# Autodesk Inventor assembly: ASY MSC 800 gills
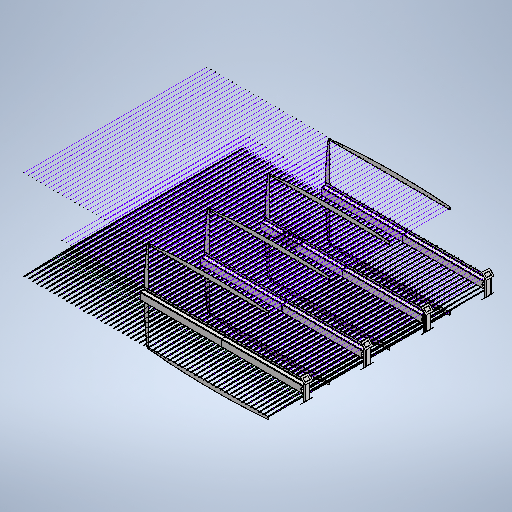
[picture p0: Inventor's stored thumbnail of the model, 512x512]
Saved by Autodesk Inventor 2025.1 (Build 291241020, 241B)
## iProperties
Created: 2024-08-31
Part Number: ASY MSC 800 gills
Document SubType Name: Assembly
Designer: pokla
Stock Number: ASY МОО 800 Жабры
Mass: 469810 g
Surface Area: 1.86943e+06 cm^2
Volume: 67870.7 cm^3
Density: 6.92212 g/cm^3
Author: pokla
## Documents named in this file (14)
- C:\Users\user\YandexDisk-badmisterfox\домашниий пк\Inventor\Manturovo\Manturovo_Se-clar\ASY MSC 800 gills.iam
- C:\Users\user\YandexDisk-badmisterfox\домашниий пк\Inventor\Manturovo\Manturovo_Se-clar\MSC 804 sheet gills.ipt
- C:\Users\user\YandexDisk-badmisterfox\домашниий пк\Inventor\Manturovo\Manturovo_Se-clar\MSC 810 pillar gills.ipt
- C:\Users\user\YandexDisk-badmisterfox\домашниий пк\Inventor\Manturovo\Manturovo_Se-clar\MSC 805 sheet gills.ipt
- C:\Users\user\YandexDisk-badmisterfox\домашниий пк\Inventor\Manturovo\Manturovo_Se-clar\MSC 806 sheet gills.ipt
- C:\Users\user\YandexDisk-badmisterfox\домашниий пк\Inventor\Manturovo\Manturovo_Se-clar\MSC 807 sheet gills.ipt
- C:\Users\user\YandexDisk-badmisterfox\домашниий пк\Inventor\Manturovo\Manturovo_Se-clar\MSC 808 sheet gills.ipt
- C:\Users\user\YandexDisk-badmisterfox\домашниий пк\Inventor\Manturovo\Manturovo_Se-clar\MSC 809 sheet gills.ipt
- C:\Users\user\YandexDisk-badmisterfox\домашниий пк\Inventor\Manturovo\Manturovo_Se-clar\MSC 813 wall support gills.ipt
- C:\Users\user\YandexDisk-badmisterfox\домашниий пк\Inventor\Manturovo\Manturovo_Se-clar\MSC 811 pillar gills.ipt
- C:\Users\user\YandexDisk-badmisterfox\домашниий пк\Inventor\Manturovo\Manturovo_Se-clar\MSC 814 string for sheets gills.ipt
- C:\Users\user\YandexDisk-badmisterfox\домашниий пк\Inventor\Manturovo\Manturovo_Se-clar\MSC 812 top support gills.ipt
- C:\Users\user\YandexDisk-badmisterfox\домашниий пк\Inventor\Manturovo\Manturovo_Se-clar\MSC 803 sheet gills.ipt
- C:\Users\user\YandexDisk-badmisterfox\домашниий пк\Inventor\Manturovo\Manturovo_Se-clar\ASY MSC 800.1 gills base.iam
## Components (393 placed, 13 different names)
1. MSC 0203 sheet gills:1 — Angle:2, Tangent:8, Tangent:9, Flush:15, Flush:19
2. MSC 0204 sheet gills:1 — Angle:3, Tangent:10, Tangent:11, Flush:15, Flush:16
3. MSC 0205 sheet gills:1 — Angle:4, Tangent:12, Tangent:13, Flush:16, Flush:17
4. MSC 0206 sheet gills:1 — Angle:5, Tangent:17, Tangent:18, Flush:17, Flush:18
5. MSC 0207 sheet gills:1 — Angle:6, Tangent:19, Tangent:20, Flush:18
6. MSC 814 string for sheets gills:143 — Rigid:40
7. MSC 0203 sheet gills:2
8. MSC 0204 sheet gills:2
9. MSC 0205 sheet gills:2
10. MSC 0206 sheet gills:2
11. MSC 0207 sheet gills:2
12. MSC 814 string for sheets gills:152 — Rigid:24
13. MSC 814 string for sheets gills:371
14. MSC 814 string for sheets gills:372
15. MSC 814 string for sheets gills:373
16. MSC 814 string for sheets gills:374
17. MSC 814 string for sheets gills:375
18. MSC 814 string for sheets gills:2 — Rigid:12
19. MSC 0201 sheet gills:1 — Rigid:33, Angle:2, Angle:3, Angle:4, Angle:5, Angle:6, Tangent:14, Tangent:15, Tangent:16, Flush:19
20. MSC 804 sheet gills:1 — Rigid:33
21. MSC 814 string for sheets gills:1 — Rotational:1
22. MSC 814 string for sheets gills:3 — Rotational:2
23. MSC 814 string for sheets gills:376 — Rotational:3
24. MSC 814 string for sheets gills:377
25. MSC 0201 sheet gills:2
26. MSC 804 sheet gills:2
27. MSC 814 string for sheets gills:378
28. MSC 814 string for sheets gills:379
29. MSC 814 string for sheets gills:380
30. MSC 814 string for sheets gills:381
31. MSC 0201 sheet gills:3
32. MSC 804 sheet gills:3
33. MSC 814 string for sheets gills:382
34. MSC 814 string for sheets gills:383
35. MSC 814 string for sheets gills:384
36. MSC 814 string for sheets gills:385
37. MSC 0201 sheet gills:4
38. MSC 804 sheet gills:4
39. MSC 814 string for sheets gills:386
40. MSC 814 string for sheets gills:387
41. MSC 814 string for sheets gills:388
42. MSC 814 string for sheets gills:389
43. MSC 0201 sheet gills:5
44. MSC 804 sheet gills:5
45. MSC 814 string for sheets gills:390
46. MSC 814 string for sheets gills:391
47. MSC 814 string for sheets gills:392
48. MSC 814 string for sheets gills:393
49. MSC 0201 sheet gills:6
50. MSC 804 sheet gills:6
51. MSC 814 string for sheets gills:394
52. MSC 814 string for sheets gills:395
53. MSC 814 string for sheets gills:396
54. MSC 814 string for sheets gills:397
55. MSC 0201 sheet gills:7
56. MSC 804 sheet gills:7
57. MSC 814 string for sheets gills:398
58. MSC 814 string for sheets gills:399
59. MSC 814 string for sheets gills:400
60. MSC 814 string for sheets gills:401
61. MSC 0201 sheet gills:8
62. MSC 804 sheet gills:8
63. MSC 814 string for sheets gills:402
64. MSC 814 string for sheets gills:403
65. MSC 814 string for sheets gills:404
66. MSC 814 string for sheets gills:405
67. MSC 0201 sheet gills:9
68. MSC 804 sheet gills:9
69. MSC 814 string for sheets gills:406
70. MSC 814 string for sheets gills:407
71. MSC 814 string for sheets gills:408
72. MSC 814 string for sheets gills:409
73. MSC 0201 sheet gills:10
74. MSC 804 sheet gills:10
75. MSC 814 string for sheets gills:410
76. MSC 814 string for sheets gills:411
77. MSC 814 string for sheets gills:412
78. MSC 814 string for sheets gills:413
79. MSC 0201 sheet gills:11
80. MSC 804 sheet gills:11
81. MSC 814 string for sheets gills:414
82. MSC 814 string for sheets gills:415
83. MSC 814 string for sheets gills:416
84. MSC 814 string for sheets gills:417
85. MSC 0201 sheet gills:12
86. MSC 804 sheet gills:12
87. MSC 814 string for sheets gills:418
88. MSC 814 string for sheets gills:419
89. MSC 814 string for sheets gills:420
90. MSC 814 string for sheets gills:421
91. MSC 0201 sheet gills:13
92. MSC 804 sheet gills:13
93. MSC 814 string for sheets gills:422
94. MSC 814 string for sheets gills:423
95. MSC 814 string for sheets gills:424
96. MSC 814 string for sheets gills:425
97. MSC 0201 sheet gills:14
98. MSC 804 sheet gills:14
99. MSC 814 string for sheets gills:426
100. MSC 814 string for sheets gills:427
101. MSC 814 string for sheets gills:428
102. MSC 814 string for sheets gills:429
103. MSC 0201 sheet gills:15
104. MSC 804 sheet gills:15
105. MSC 814 string for sheets gills:430
106. MSC 814 string for sheets gills:431
107. MSC 814 string for sheets gills:432
108. MSC 814 string for sheets gills:433
109. MSC 0201 sheet gills:16
110. MSC 804 sheet gills:16
111. MSC 814 string for sheets gills:434
112. MSC 814 string for sheets gills:435
113. MSC 814 string for sheets gills:436
114. MSC 814 string for sheets gills:437
115. MSC 0201 sheet gills:17
116. MSC 804 sheet gills:17
117. MSC 814 string for sheets gills:438
118. MSC 814 string for sheets gills:439
119. MSC 814 string for sheets gills:440
120. MSC 814 string for sheets gills:441
121. MSC 0201 sheet gills:18
122. MSC 804 sheet gills:18
123. MSC 814 string for sheets gills:442
124. MSC 814 string for sheets gills:443
125. MSC 814 string for sheets gills:444
126. MSC 814 string for sheets gills:445
127. MSC 0201 sheet gills:19
128. MSC 804 sheet gills:19
129. MSC 814 string for sheets gills:446
130. MSC 814 string for sheets gills:447
131. MSC 814 string for sheets gills:448
132. MSC 814 string for sheets gills:449
133. MSC 0201 sheet gills:20
134. MSC 804 sheet gills:20
135. MSC 814 string for sheets gills:450
136. MSC 814 string for sheets gills:451
137. MSC 814 string for sheets gills:452
138. MSC 814 string for sheets gills:453
139. MSC 0201 sheet gills:21
140. MSC 804 sheet gills:21
141. MSC 814 string for sheets gills:454
142. MSC 814 string for sheets gills:455
143. MSC 814 string for sheets gills:456
144. MSC 814 string for sheets gills:457
145. MSC 0201 sheet gills:22
146. MSC 804 sheet gills:22
147. MSC 814 string for sheets gills:458
148. MSC 814 string for sheets gills:459
149. MSC 814 string for sheets gills:460
150. MSC 814 string for sheets gills:461
151. MSC 0201 sheet gills:23
152. MSC 804 sheet gills:23
153. MSC 814 string for sheets gills:462
154. MSC 814 string for sheets gills:463
155. MSC 814 string for sheets gills:464
156. MSC 814 string for sheets gills:465
157. MSC 0201 sheet gills:24
158. MSC 804 sheet gills:24
159. MSC 814 string for sheets gills:466
160. MSC 814 string for sheets gills:467
161. MSC 814 string for sheets gills:468
162. MSC 814 string for sheets gills:469
163. MSC 0201 sheet gills:25
164. MSC 804 sheet gills:25
165. MSC 814 string for sheets gills:470
166. MSC 814 string for sheets gills:471
167. MSC 814 string for sheets gills:472
168. MSC 814 string for sheets gills:473
169. MSC 0201 sheet gills:26
170. MSC 804 sheet gills:26
171. MSC 814 string for sheets gills:474
172. MSC 814 string for sheets gills:475
173. MSC 814 string for sheets gills:476
174. MSC 814 string for sheets gills:477
175. MSC 0201 sheet gills:27
176. MSC 804 sheet gills:27
177. MSC 814 string for sheets gills:478
178. MSC 814 string for sheets gills:479
179. MSC 814 string for sheets gills:480
180. MSC 814 string for sheets gills:481
181. MSC 0201 sheet gills:28
182. MSC 804 sheet gills:28
183. MSC 814 string for sheets gills:482
184. MSC 814 string for sheets gills:483
185. MSC 814 string for sheets gills:484
186. MSC 814 string for sheets gills:485
187. MSC 0201 sheet gills:29
188. MSC 804 sheet gills:29
189. MSC 814 string for sheets gills:486
190. MSC 814 string for sheets gills:487
191. MSC 814 string for sheets gills:488
192. MSC 814 string for sheets gills:489
193. MSC 0201 sheet gills:30
194. MSC 804 sheet gills:30
195. MSC 814 string for sheets gills:490
196. MSC 814 string for sheets gills:491
197. MSC 814 string for sheets gills:492
198. MSC 814 string for sheets gills:493
199. MSC 0201 sheet gills:31
200. MSC 804 sheet gills:31
201. MSC 814 string for sheets gills:494
202. MSC 814 string for sheets gills:495
203. MSC 814 string for sheets gills:496
204. MSC 814 string for sheets gills:497
205. MSC 0201 sheet gills:32
206. MSC 804 sheet gills:32
207. MSC 814 string for sheets gills:498
208. MSC 814 string for sheets gills:499
209. MSC 814 string for sheets gills:500
210. MSC 814 string for sheets gills:501
211. MSC 0201 sheet gills:33
212. MSC 804 sheet gills:33
213. MSC 814 string for sheets gills:502
214. MSC 814 string for sheets gills:503
215. MSC 814 string for sheets gills:504
216. MSC 814 string for sheets gills:505
217. MSC 0201 sheet gills:34
218. MSC 804 sheet gills:34
219. MSC 814 string for sheets gills:506
220. MSC 814 string for sheets gills:507
221. MSC 814 string for sheets gills:508
222. MSC 814 string for sheets gills:509
223. MSC 0201 sheet gills:35
224. MSC 804 sheet gills:35
225. MSC 814 string for sheets gills:510
226. MSC 814 string for sheets gills:511
227. MSC 814 string for sheets gills:512
228. MSC 814 string for sheets gills:513
229. MSC 0201 sheet gills:36
230. MSC 804 sheet gills:36
231. MSC 814 string for sheets gills:514
232. MSC 814 string for sheets gills:515
233. MSC 814 string for sheets gills:516
234. MSC 814 string for sheets gills:517
235. MSC 0201 sheet gills:37
236. MSC 804 sheet gills:37
237. MSC 814 string for sheets gills:518
238. MSC 814 string for sheets gills:519
239. MSC 814 string for sheets gills:520
240. MSC 814 string for sheets gills:521
241. MSC 0201 sheet gills:38
242. MSC 804 sheet gills:38
243. MSC 814 string for sheets gills:522
244. MSC 814 string for sheets gills:523
245. MSC 814 string for sheets gills:524
246. MSC 814 string for sheets gills:525
247. MSC 0201 sheet gills:39
248. MSC 804 sheet gills:39
249. MSC 814 string for sheets gills:526
250. MSC 814 string for sheets gills:527
251. MSC 814 string for sheets gills:528
252. MSC 814 string for sheets gills:529
253. MSC 0201 sheet gills:40
254. MSC 804 sheet gills:40
255. MSC 814 string for sheets gills:530
256. MSC 814 string for sheets gills:531
257. MSC 814 string for sheets gills:532
258. MSC 814 string for sheets gills:533
259. MSC 0201 sheet gills:41
260. MSC 804 sheet gills:41
261. MSC 814 string for sheets gills:534
262. MSC 814 string for sheets gills:535
263. MSC 814 string for sheets gills:536
264. MSC 814 string for sheets gills:537
265. MSC 0201 sheet gills:42
266. MSC 804 sheet gills:42
267. MSC 814 string for sheets gills:538
268. MSC 814 string for sheets gills:539
269. MSC 814 string for sheets gills:540
270. MSC 814 string for sheets gills:541
271. MSC 0201 sheet gills:43
272. MSC 804 sheet gills:43
273. MSC 814 string for sheets gills:542
274. MSC 814 string for sheets gills:543
275. MSC 814 string for sheets gills:544
276. MSC 814 string for sheets gills:545
277. MSC 0201 sheet gills:44
278. MSC 804 sheet gills:44
279. MSC 814 string for sheets gills:546
280. MSC 814 string for sheets gills:547
281. MSC 814 string for sheets gills:548
282. MSC 814 string for sheets gills:549
283. MSC 0201 sheet gills:45
284. MSC 804 sheet gills:45
285. MSC 814 string for sheets gills:550
286. MSC 814 string for sheets gills:551
287. MSC 814 string for sheets gills:552
288. MSC 814 string for sheets gills:553
289. MSC 0201 sheet gills:46
290. MSC 804 sheet gills:46
291. MSC 814 string for sheets gills:554
292. MSC 814 string for sheets gills:555
293. MSC 814 string for sheets gills:556
294. MSC 814 string for sheets gills:557
295. MSC 0201 sheet gills:47
296. MSC 804 sheet gills:47
297. MSC 814 string for sheets gills:558
298. MSC 814 string for sheets gills:559
299. MSC 814 string for sheets gills:560
300. MSC 814 string for sheets gills:561
301. MSC 0201 sheet gills:48
302. MSC 804 sheet gills:48
303. MSC 814 string for sheets gills:562
304. MSC 814 string for sheets gills:563
305. MSC 814 string for sheets gills:564
306. MSC 814 string for sheets gills:565
307. MSC 0201 sheet gills:49
308. MSC 804 sheet gills:49
309. MSC 814 string for sheets gills:566
310. MSC 814 string for sheets gills:567
311. MSC 814 string for sheets gills:568
312. MSC 814 string for sheets gills:569
313. MSC 0201 sheet gills:50
314. MSC 804 sheet gills:50
315. MSC 814 string for sheets gills:570
316. MSC 814 string for sheets gills:571
317. MSC 814 string for sheets gills:572
318. MSC 814 string for sheets gills:573
319. MSC 0201 sheet gills:51
320. MSC 804 sheet gills:51
321. MSC 814 string for sheets gills:574
322. MSC 814 string for sheets gills:575
323. MSC 814 string for sheets gills:576
324. MSC 814 string for sheets gills:577
325. MSC 0201 sheet gills:52
326. MSC 804 sheet gills:52
327. MSC 814 string for sheets gills:578
328. MSC 814 string for sheets gills:579
329. MSC 814 string for sheets gills:580
330. MSC 814 string for sheets gills:581
331. MSC 0201 sheet gills:53
332. MSC 804 sheet gills:53
333. MSC 814 string for sheets gills:582
334. MSC 814 string for sheets gills:583
335. MSC 814 string for sheets gills:584
336. MSC 814 string for sheets gills:585
337. MSC 0201 sheet gills:54
338. MSC 804 sheet gills:54
339. MSC 814 string for sheets gills:586
340. MSC 814 string for sheets gills:587
341. MSC 814 string for sheets gills:588
342. MSC 814 string for sheets gills:589
343. MSC 0201 sheet gills:55
344. MSC 804 sheet gills:55
345. MSC 814 string for sheets gills:590
346. MSC 814 string for sheets gills:591
347. MSC 814 string for sheets gills:592
348. MSC 814 string for sheets gills:593
349. MSC 0201 sheet gills:56
350. MSC 804 sheet gills:56
351. MSC 814 string for sheets gills:594
352. MSC 814 string for sheets gills:595
353. MSC 814 string for sheets gills:596
354. MSC 814 string for sheets gills:597
355. MSC 0201 sheet gills:57
356. MSC 804 sheet gills:57
357. MSC 814 string for sheets gills:598
358. MSC 814 string for sheets gills:599
359. MSC 814 string for sheets gills:600
360. MSC 814 string for sheets gills:601
361. MSC 0201 sheet gills:58
362. MSC 804 sheet gills:58
363. MSC 814 string for sheets gills:602
364. MSC 814 string for sheets gills:603
365. MSC 814 string for sheets gills:604
366. MSC 813 wall support gills:1 — Rigid:12, Rigid:30, Tangent:14, Tangent:15
367. MSC 812 top support gills:1 — Rigid:28, Rigid:30, Tangent:8, Tangent:9, Tangent:10, Tangent:11, Tangent:12, Tangent:13, Tangent:17, Tangent:18, Tangent:19, Tangent:20, Rigid:40
368. MSC 811 pillar gills:1 — Rigid:28, Rigid:29
369. MSC 812 top support gills:2 — Rigid:24, Rigid:29, Rigid:31
370. MSC 813 wall support gills:2 — Rigid:31, Rotational:3
371. MSC 810 pillar gills:1 — Rotational:1, Rotational:2, Tangent:16
372. ASY MSC 800.1 gills base:1 [sub-assembly]
373. MSC 813 wall support gills:4
374. MSC 812 top support gills:3
375. MSC 811 pillar gills:2
376. MSC 812 top support gills:4
377. MSC 813 wall support gills:5
378. MSC 810 pillar gills:2
379. ASY MSC 800.1 gills base:2 [sub-assembly]
380. MSC 813 wall support gills:6
381. MSC 812 top support gills:5
382. MSC 811 pillar gills:3
383. MSC 812 top support gills:6
384. MSC 813 wall support gills:7
385. MSC 810 pillar gills:3
386. ASY MSC 800.1 gills base:3 [sub-assembly]
387. MSC 813 wall support gills:8
388. MSC 812 top support gills:7
389. MSC 811 pillar gills:4
390. MSC 812 top support gills:8
391. MSC 813 wall support gills:9
392. MSC 810 pillar gills:4
393. ASY MSC 800.1 gills base:4 [sub-assembly]
## Component patterns: (6 elements, first: MSC 814 string for sheets gills:152), (58 elements, first: MSC 814 string for sheets gills:2 + MSC 0201 sheet gills:1 + MSC 804 sheet gills:1 + MSC 814 string for sheets gills:1 + MSC 814 string for sheets gills:3 + MSC 814 string for sheets gills:376), (4 elements, first: MSC 813 wall support gills:1 + MSC 812 top support gills:1 + MSC 811 pillar gills:1 + MSC 812 top support gills:2 + MSC 813 wall support gills:2 + MSC 810 pillar gills:1 + ASY MSC 800.1 gills base:1)
## Relationships (45: Tangent 13, Flush 12, WeldJoint 9, Angle 5, Mate 3, RevoluteJoint 3)
- [WeldJoint]: MSC 811 pillar gills:1 ↔ MSC 810 pillar gills:1
- [Flush]: MSC 810 pillar gills:1 ↔ ASY MSC 800.1 gills base:1
- [Mate]: MSC 810 pillar gills:1 ↔ ASY MSC 800.1 gills base:1
- [Flush] (5 mm): MSC 810 pillar gills:1 ↔ ASY MSC 800.1 gills base:1
- Rigid:12 [WeldJoint] (-5 mm): MSC 814 string for sheets gills:2 ↔ MSC 813 wall support gills:1
- [Mate]: ASY MSC 800.1 gills base:1
- [Mate]: ASY MSC 800.1 gills base:1
- [Flush]: ASY MSC 800.1 gills base:1
- Rigid:24 [WeldJoint] (-5 mm): MSC 814 string for sheets gills:152 ↔ MSC 812 top support gills:2
- Rigid:28 [WeldJoint]: MSC 812 top support gills:1 ↔ MSC 811 pillar gills:1
- Rigid:29 [WeldJoint]: MSC 811 pillar gills:1 ↔ MSC 812 top support gills:2
- Rigid:30 [WeldJoint]: MSC 813 wall support gills:1 ↔ MSC 812 top support gills:1
- Rigid:31 [WeldJoint]: MSC 812 top support gills:2 ↔ MSC 813 wall support gills:2
- Rotational:1 [RevoluteJoint] (5 mm): MSC 814 string for sheets gills:1 ↔ MSC 810 pillar gills:1
- Rotational:2 [RevoluteJoint] (-5 mm): MSC 814 string for sheets gills:3 ↔ MSC 810 pillar gills:1
- Rigid:33 [WeldJoint] (-10 mm): MSC 0201 sheet gills:1 ↔ MSC 804 sheet gills:1
- Angle:2 (0 deg): MSC 0203 sheet gills:1 ↔ MSC 0201 sheet gills:1
- Angle:3 (0 deg): MSC 0204 sheet gills:1 ↔ MSC 0201 sheet gills:1
- Angle:4 (0 deg): MSC 0205 sheet gills:1 ↔ MSC 0201 sheet gills:1
- Angle:5 (0 deg): MSC 0206 sheet gills:1 ↔ MSC 0201 sheet gills:1
- Angle:6 (0 deg): MSC 0207 sheet gills:1 ↔ MSC 0201 sheet gills:1
- Tangent:8: MSC 0203 sheet gills:1 ↔ MSC 812 top support gills:1
- Tangent:9: MSC 0203 sheet gills:1 ↔ MSC 812 top support gills:1
- Tangent:10: MSC 0204 sheet gills:1 ↔ MSC 812 top support gills:1
- Tangent:11: MSC 0204 sheet gills:1 ↔ MSC 812 top support gills:1
- Tangent:12: MSC 0205 sheet gills:1 ↔ MSC 812 top support gills:1
- Tangent:13: MSC 0205 sheet gills:1 ↔ MSC 812 top support gills:1
- Tangent:14: MSC 0201 sheet gills:1 ↔ MSC 813 wall support gills:1
- Tangent:15: MSC 0201 sheet gills:1 ↔ MSC 813 wall support gills:1
- Tangent:16: MSC 0201 sheet gills:1 ↔ MSC 810 pillar gills:1
- Tangent:17: MSC 0206 sheet gills:1 ↔ MSC 812 top support gills:1
- Tangent:18: MSC 0206 sheet gills:1 ↔ MSC 812 top support gills:1
- Tangent:19: MSC 0207 sheet gills:1 ↔ MSC 812 top support gills:1
- Tangent:20: MSC 0207 sheet gills:1 ↔ MSC 812 top support gills:1
- Flush:15: MSC 0203 sheet gills:1 ↔ MSC 0204 sheet gills:1
- Flush:16: MSC 0204 sheet gills:1 ↔ MSC 0205 sheet gills:1
- Flush:17: MSC 0205 sheet gills:1 ↔ MSC 0206 sheet gills:1
- Flush:18: MSC 0206 sheet gills:1 ↔ MSC 0207 sheet gills:1
- Flush:19: MSC 0203 sheet gills:1 ↔ MSC 0201 sheet gills:1
- Rigid:40 [WeldJoint] (5 mm): MSC 814 string for sheets gills:143 ↔ MSC 812 top support gills:1
- Rotational:3 [RevoluteJoint] (-5 mm): MSC 814 string for sheets gills:376 ↔ MSC 813 wall support gills:2
- [Flush]: MSC 0203 sheet gills:2 ↔ MSC 0204 sheet gills:2
- [Flush]: MSC 0204 sheet gills:2 ↔ MSC 0205 sheet gills:2
- [Flush]: MSC 0205 sheet gills:2 ↔ MSC 0206 sheet gills:2
- [Flush]: MSC 0206 sheet gills:2 ↔ MSC 0207 sheet gills:2
## Named parameters: d265_d202 = 0 mm, d266_d203 = 0 mm, d267_d204 = 0 mm, d268_d205 = 0 mm
